# Autodesk Inventor assembly: SecondAssembly
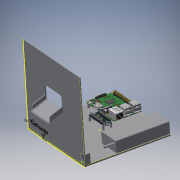
[picture p0: Inventor's stored thumbnail of the model, 180x180]
Saved by Autodesk Inventor 2019 (Build 230136000, 136)
## iProperties
Created: 2018-12-20
Part Number: SecondAssembly
Document SubType Name: Assembly
Designer: assman
Author: assman
## Documents named in this file (5)
- D:\Inventor\CatFeeder\tests\SecondAssembly.iam
- D:\Inventor\CatFeeder\ArduinoNano\arduino nano.iam
- D:\Inventor\CatFeeder\Raspberry Pi 3.ipt
- D:\Inventor\CatFeeder\Enclosure.ipt
- D:\Inventor\CatFeeder\Transformer.ipt
## Components (4 placed, 4 different names)
1. Raspberry Pi 3:1
2. Enclosure:1 — Rigid:2, Rigid:3
3. Transformer:1 — Rigid:3
4. arduino nano:1 [sub-assembly] — Rigid:2
## Relationships (2: WeldJoint 2)
- Rigid:2 [WeldJoint]: Enclosure:1 ↔ arduino nano:1
- Rigid:3 [WeldJoint]: Enclosure:1 ↔ Transformer:1
